# Autodesk Inventor assembly: Spool
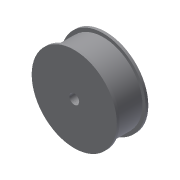
[picture p0: Inventor's stored thumbnail of the model, 180x180]
Saved by Autodesk Inventor 2015 (Build 190159000, 159)
## iProperties
Created: 2015-03-09
Part Number: Spool
Document SubType Name: Assembly
Designer: Jaden
Author: Jaden
## Documents named in this file (3)
- E:\ReDesign\Spool.iam
- E:\ReDesign\spoolmain.ipt
- E:\ReDesign\SpoolGuard.ipt
## Components (3 placed, 2 different names)
1. spoolmain:1 — Mate:1, Mate:2, Mate:3, Mate:4
2. SpoolGuard:1 — Mate:3, Mate:4
3. SpoolGuard:2 — Mate:1, Mate:2
## Relationships (4: Mate 4)
- Mate:1: spoolmain:1 ↔ SpoolGuard:2
- Mate:2: spoolmain:1 ↔ SpoolGuard:2
- Mate:3: spoolmain:1 ↔ SpoolGuard:1
- Mate:4: spoolmain:1 ↔ SpoolGuard:1
